# Autodesk Inventor assembly: Casing
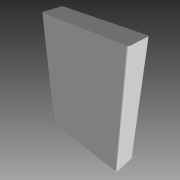
[picture p0: Inventor's stored thumbnail of the model, 180x180]
Saved by Autodesk Inventor 2016 (Build 200138000, 138)
## iProperties
Created: 2015-03-25
Part Number: Casing
Document SubType Name: Assembly
Designer: Yann
Author: Yann
## Documents named in this file (3)
- C:\Users\Yann\Documents\GitHub\BIKAIR_CAD\Source\Energy_Pack\Casing.iam
- C:\Users\Yann\Documents\GitHub\BIKAIR_CAD\Source\Energy_Pack\Casing_Generator.ipt
- C:\Users\Yann\Documents\GitHub\BIKAIR_CAD\Source\Temp\11.ipt
## Components (2 placed, 2 different names)
1. Casing_Generator:1 — Placage:1, Placage:2, Affleurement:1
2. 11:1 — Placage:4, Placage:5
## Relationships (5: Mate 4, Flush 1)
- Placage:1 [Mate]: Casing_Generator:1
- Placage:2 [Mate]: Casing_Generator:1
- Affleurement:1 [Flush]: Casing_Generator:1
- Placage:4 [Mate]: 11:1
- Placage:5 [Mate]: 11:1
